# Autodesk Inventor assembly: full_layout_test
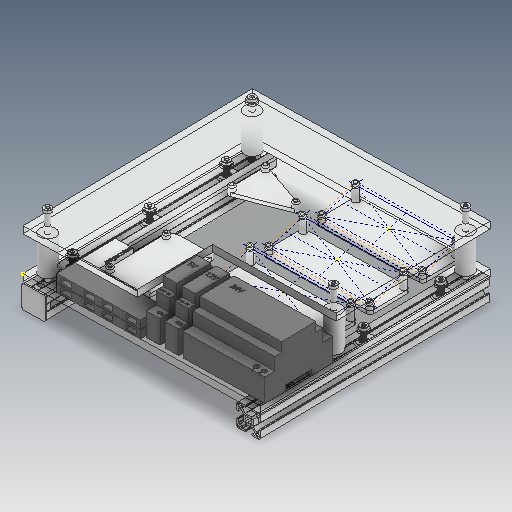
[picture p0: Inventor's stored thumbnail of the model, 512x512]
Saved by Autodesk Inventor 2025.4 (Build 294407020, 407B)
## iProperties
Created: 2026-09-08
Part Number: full_layout_test
Document SubType Name: Assembly
Designer: Aiden
Author: Aiden
## Documents named in this file (19)
- C:\Users\Aiden\Documents\GitHub\coldex-instrumentation\3d_models\mounting_hardware\dummy_parts\full_layout_test.iam
- C:\Users\Aiden\Documents\GitHub\coldex-instrumentation\3d_models\mounting_hardware\dummy_parts\acrylic_base.ipt
- C:\Users\Aiden\Documents\GitHub\coldex-instrumentation\3d_models\mounting_hardware\dummy_parts\acrylic_cover.ipt
- C:\Users\Aiden\Documents\GitHub\coldex-instrumentation\3d_models\mounting_hardware\McMaster\30mm_1ft_T-Slotted Framing.ipt
- C:\Users\Aiden\Documents\GitHub\coldex-instrumentation\3d_models\mounting_hardware\McMaster\30mm_teenut_T-Slotted Framing.ipt
- C:\Users\Aiden\Documents\GitHub\coldex-instrumentation\3d_models\mounting_hardware\McMaster\0.257in_innerD_Moisture-Resistant Cushioning Washer.ipt
- C:\Users\Aiden\Documents\GitHub\coldex-instrumentation\3d_models\mounting_hardware\McMaster\m6_18mm_18-8 Stainless Steel Low-Profile Socket Head Screws.ipt
- C:\Users\Aiden\Documents\GitHub\coldex-instrumentation\3d_models\mounting_hardware\dummy_parts\din_rail.ipt
- C:\Users\Aiden\Documents\GitHub\coldex-instrumentation\3d_models\mounting_hardware\dummy_parts\5V_din_voltage_regulator.ipt
- C:\Users\Aiden\Documents\GitHub\coldex-instrumentation\3d_models\mounting_hardware\dummy_parts\12V_din_voltage_regulator.ipt
- C:\Users\Aiden\Documents\GitHub\coldex-instrumentation\3d_models\mounting_hardware\dummy_parts\24V_din_pwr_supply.ipt
- C:\Users\Aiden\Documents\GitHub\coldex-instrumentation\3d_models\mounting_hardware\relay_module_standoffs_angled_plate.ipt
- C:\Users\Aiden\Documents\GitHub\coldex-instrumentation\3d_models\mounting_hardware\arduino_mega_standoffs_plate.ipt
- C:\Users\Aiden\Documents\GitHub\coldex-instrumentation\3d_models\mounting_hardware\dummy_parts\adalogger_mcu_volume.ipt
- C:\Users\Aiden\Documents\GitHub\coldex-instrumentation\3d_models\mounting_hardware\db-25_standoffs_plate.ipt
- C:\Users\Aiden\Documents\GitHub\coldex-instrumentation\3d_models\mounting_hardware\dummy_parts\anker_4-port_usb3.0_splitter.ipt
- C:\Users\Aiden\Documents\GitHub\coldex-instrumentation\3d_models\mounting_hardware\dummy_parts\spacer_temp.ipt
- C:\Users\Aiden\Documents\GitHub\coldex-instrumentation\3d_models\mounting_hardware\McMaster\m6_70mm_18-8 Stainless Steel Low-Profile Socket Head Screws.ipt
- C:\Users\Aiden\Documents\GitHub\coldex-instrumentation\3d_models\mounting_hardware\dummy_parts\8020_Cap.ipt
## Components (44 placed, 18 different names)
1. acrylic_base:1 — Flush:1, Flush:2, Mate:1, Mate:2, Flush:3, Flush:4, Mate:9, Mate:10, Mate:11, Mate:12, Mate:13, Mate:14, Mate:21, Mate:22, Mate:23, Mate:24, Mate:25, Mate:26, Mate:39, Mate:47, Angle:1, Flush:6, Mate:48, Angle:2, Angle:3, Mate:49, Mate:50, Angle:4, Mate:51, Flush:7, Mate:53, Mate:54, Mate:55, Mate:56, Mate:57, Mate:58, Mate:59, Mate:60
2. acrylic_cover:1 — Flush:1, Flush:2, Mate:61, Mate:62, Mate:63, Mate:64, Mate:65, Mate:67
3. 30mm_1ft_T-Slotted Framing:1 — Mate:1, Flush:4, Mate:3, Mate:4, Mate:5, Tangent:2, Flush:10
4. 30mm_1ft_T-Slotted Framing:2 — Mate:2, Flush:3, Mate:6, Mate:7, Mate:8, Tangent:1, Flush:5
5. 30mm_teenut_T-Slotted Framing:1 — Mate:5, Mate:9
6. 30mm_teenut_T-Slotted Framing:2 — Mate:3, Mate:10
7. 30mm_teenut_T-Slotted Framing:3 — Mate:4, Mate:11, Tangent:2
8. 30mm_teenut_T-Slotted Framing:4 — Mate:7, Mate:13
9. 30mm_teenut_T-Slotted Framing:5 — Mate:6, Mate:14
10. 30mm_teenut_T-Slotted Framing:6 — Mate:8, Mate:12, Tangent:1
11. m6_18mm_18-8 Stainless Steel Low-Profile Socket Head Screws:1 — Mate:35
12. m6_18mm_18-8 Stainless Steel Low-Profile Socket Head Screws:2 — Mate:34
13. m6_18mm_18-8 Stainless Steel Low-Profile Socket Head Screws:3
14. m6_18mm_18-8 Stainless Steel Low-Profile Socket Head Screws:4 — Mate:36
15. m6_18mm_18-8 Stainless Steel Low-Profile Socket Head Screws:5 — Mate:37
16. m6_18mm_18-8 Stainless Steel Low-Profile Socket Head Screws:6 — Mate:38, Mate:40
17. 0.257in_innerD_Moisture-Resistant Cushioning Washer:1 — Mate:22, Mate:34
18. 0.257in_innerD_Moisture-Resistant Cushioning Washer:2 — Mate:23, Mate:35
19. 0.257in_innerD_Moisture-Resistant Cushioning Washer:3 — Mate:24, Mate:38
20. 0.257in_innerD_Moisture-Resistant Cushioning Washer:4 — Mate:26, Mate:36
21. 0.257in_innerD_Moisture-Resistant Cushioning Washer:5 — Mate:25, Mate:37
22. 0.257in_innerD_Moisture-Resistant Cushioning Washer:6 — Mate:21
23. din_rail:1 — Mate:39, Mate:40, Mate:41, Mate:42, Mate:43, Mate:44, Mate:45, Mate:46
24. 5V_din_voltage_regulator:1 — Mate:41, Mate:42
25. 12V_din_voltage_regulator:1 — Mate:43, Mate:44
26. 24V_din_pwr_supply:1 — Mate:45, Mate:46
27. arduino_mega_standoffs_plate:1 — Angle:3, Mate:49
28. adalogger_mcu_volume:1 — Mate:48, Angle:2
29. db-25_standoffs_plate:1 — Mate:50, Angle:4
30. anker_4-port_usb3.0_splitter:1 — Mate:51, Flush:7, Flush:8, Mate:52, Flush:9
31. anker_4-port_usb3.0_splitter:2 — Flush:8, Mate:52, Flush:9
32. spacer_temp:1 — Mate:53, Mate:58
33. spacer_temp:2 — Mate:54, Mate:60
34. spacer_temp:3 — Mate:56, Mate:59
35. spacer_temp:4 — Mate:55, Mate:57, Mate:61
36. m6_70mm_18-8 Stainless Steel Low-Profile Socket Head Screws:1 — Mate:62, Mate:66, Mate:68
37. m6_70mm_18-8 Stainless Steel Low-Profile Socket Head Screws:2 — Mate:63
38. m6_70mm_18-8 Stainless Steel Low-Profile Socket Head Screws:3 — Mate:64
39. m6_70mm_18-8 Stainless Steel Low-Profile Socket Head Screws:4 — Mate:65
40. 0.257in_innerD_Moisture-Resistant Cushioning Washer:7 — Mate:66, Mate:67, Mate:68
41. 8020_Cap:1 — Flush:10
42. relay_module_standoffs_angled_plate:1 — Mate:47, Angle:1, Flush:6
43. relay_module_standoffs_angled_plate:2 — Flush:5
44. relay_module_standoffs_angled_plate:3
## Component patterns: (3 elements, first: relay_module_standoffs_angled_plate:1)
## Relationships (84: Mate 68, Flush 10, Angle 4, Tangent 2)
- Flush:1: acrylic_base:1 ↔ acrylic_cover:1
- Flush:2: acrylic_base:1 ↔ acrylic_cover:1
- Mate:1: acrylic_base:1 ↔ 30mm_1ft_T-Slotted Framing:1
- Mate:2: acrylic_base:1 ↔ 30mm_1ft_T-Slotted Framing:2
- Flush:3: acrylic_base:1 ↔ 30mm_1ft_T-Slotted Framing:2
- Flush:4: acrylic_base:1 ↔ 30mm_1ft_T-Slotted Framing:1
- Mate:3: 30mm_1ft_T-Slotted Framing:1 ↔ 30mm_teenut_T-Slotted Framing:2
- Mate:4: 30mm_1ft_T-Slotted Framing:1 ↔ 30mm_teenut_T-Slotted Framing:3
- Mate:5: 30mm_1ft_T-Slotted Framing:1 ↔ 30mm_teenut_T-Slotted Framing:1
- Mate:6: 30mm_1ft_T-Slotted Framing:2 ↔ 30mm_teenut_T-Slotted Framing:5
- Mate:7: 30mm_1ft_T-Slotted Framing:2 ↔ 30mm_teenut_T-Slotted Framing:4
- Mate:8: 30mm_1ft_T-Slotted Framing:2 ↔ 30mm_teenut_T-Slotted Framing:6
- Mate:9: acrylic_base:1 ↔ 30mm_teenut_T-Slotted Framing:1
- Mate:10: acrylic_base:1 ↔ 30mm_teenut_T-Slotted Framing:2
- Mate:11: acrylic_base:1 ↔ 30mm_teenut_T-Slotted Framing:3
- Mate:12: acrylic_base:1 ↔ 30mm_teenut_T-Slotted Framing:6
- Mate:13: acrylic_base:1 ↔ 30mm_teenut_T-Slotted Framing:4
- Mate:14: acrylic_base:1 ↔ 30mm_teenut_T-Slotted Framing:5
- Tangent:1: 30mm_1ft_T-Slotted Framing:2 ↔ 30mm_teenut_T-Slotted Framing:6
- Tangent:2: 30mm_1ft_T-Slotted Framing:1 ↔ 30mm_teenut_T-Slotted Framing:3
- [Mate]: acrylic_base:1 ↔ m6_18mm_18-8 Stainless Steel Low-Profile Socket Head Screws:1
- [Mate]: acrylic_base:1 ↔ m6_18mm_18-8 Stainless Steel Low-Profile Socket Head Screws:2
- [Mate]: acrylic_base:1 ↔ m6_18mm_18-8 Stainless Steel Low-Profile Socket Head Screws:3
- [Mate]: acrylic_base:1 ↔ m6_18mm_18-8 Stainless Steel Low-Profile Socket Head Screws:4
- [Mate]: acrylic_base:1 ↔ m6_18mm_18-8 Stainless Steel Low-Profile Socket Head Screws:5
- [Mate]: acrylic_base:1 ↔ m6_18mm_18-8 Stainless Steel Low-Profile Socket Head Screws:6
- Mate:21: acrylic_base:1 ↔ 0.257in_innerD_Moisture-Resistant Cushioning Washer:6
- Mate:22: acrylic_base:1 ↔ 0.257in_innerD_Moisture-Resistant Cushioning Washer:1
- Mate:23: acrylic_base:1 ↔ 0.257in_innerD_Moisture-Resistant Cushioning Washer:2
- Mate:24: acrylic_base:1 ↔ 0.257in_innerD_Moisture-Resistant Cushioning Washer:3
- Mate:25: acrylic_base:1 ↔ 0.257in_innerD_Moisture-Resistant Cushioning Washer:5
- Mate:26: acrylic_base:1 ↔ 0.257in_innerD_Moisture-Resistant Cushioning Washer:4
- [Mate]: m6_18mm_18-8 Stainless Steel Low-Profile Socket Head Screws:3 ↔ 0.257in_innerD_Moisture-Resistant Cushioning Washer:6
- [Mate]: m6_18mm_18-8 Stainless Steel Low-Profile Socket Head Screws:2 ↔ 0.257in_innerD_Moisture-Resistant Cushioning Washer:1
- [Mate]: m6_18mm_18-8 Stainless Steel Low-Profile Socket Head Screws:1 ↔ 0.257in_innerD_Moisture-Resistant Cushioning Washer:2
- [Mate]: m6_18mm_18-8 Stainless Steel Low-Profile Socket Head Screws:6 ↔ 0.257in_innerD_Moisture-Resistant Cushioning Washer:3
- [Mate]: m6_18mm_18-8 Stainless Steel Low-Profile Socket Head Screws:5 ↔ 0.257in_innerD_Moisture-Resistant Cushioning Washer:5
- [Mate]: m6_18mm_18-8 Stainless Steel Low-Profile Socket Head Screws:4 ↔ 0.257in_innerD_Moisture-Resistant Cushioning Washer:4
- [Mate]: m6_18mm_18-8 Stainless Steel Low-Profile Socket Head Screws:3 ↔ 0.257in_innerD_Moisture-Resistant Cushioning Washer:6
- Mate:34: m6_18mm_18-8 Stainless Steel Low-Profile Socket Head Screws:2 ↔ 0.257in_innerD_Moisture-Resistant Cushioning Washer:1
- Mate:35: m6_18mm_18-8 Stainless Steel Low-Profile Socket Head Screws:1 ↔ 0.257in_innerD_Moisture-Resistant Cushioning Washer:2
- Mate:36: m6_18mm_18-8 Stainless Steel Low-Profile Socket Head Screws:4 ↔ 0.257in_innerD_Moisture-Resistant Cushioning Washer:4
- Mate:37: m6_18mm_18-8 Stainless Steel Low-Profile Socket Head Screws:5 ↔ 0.257in_innerD_Moisture-Resistant Cushioning Washer:5
- Mate:38: m6_18mm_18-8 Stainless Steel Low-Profile Socket Head Screws:6 ↔ 0.257in_innerD_Moisture-Resistant Cushioning Washer:3
- Mate:39: acrylic_base:1 ↔ din_rail:1
- Mate:40: m6_18mm_18-8 Stainless Steel Low-Profile Socket Head Screws:6 ↔ din_rail:1
- Mate:41: din_rail:1 ↔ 5V_din_voltage_regulator:1
- Mate:42: din_rail:1 ↔ 5V_din_voltage_regulator:1
- Mate:43: din_rail:1 ↔ 12V_din_voltage_regulator:1
- Mate:44: din_rail:1 ↔ 12V_din_voltage_regulator:1
- Mate:45: din_rail:1 ↔ 24V_din_pwr_supply:1
- Mate:46: din_rail:1 ↔ 24V_din_pwr_supply:1
- Mate:47: acrylic_base:1 ↔ relay_module_standoffs_angled_plate:1
- Angle:1 (0 deg): acrylic_base:1 ↔ relay_module_standoffs_angled_plate:1
- Flush:5 (27 mm): 30mm_1ft_T-Slotted Framing:2 ↔ relay_module_standoffs_angled_plate:2
- Flush:6 (7.5 mm): acrylic_base:1 ↔ relay_module_standoffs_angled_plate:1
- Mate:48: acrylic_base:1 ↔ adalogger_mcu_volume:1
- Angle:2 (0 deg): acrylic_base:1 ↔ adalogger_mcu_volume:1
- Angle:3 (0 deg): acrylic_base:1 ↔ arduino_mega_standoffs_plate:1
- Mate:49: acrylic_base:1 ↔ arduino_mega_standoffs_plate:1
- Mate:50: acrylic_base:1 ↔ db-25_standoffs_plate:1
- Angle:4 (0 deg): acrylic_base:1 ↔ db-25_standoffs_plate:1
- Mate:51: acrylic_base:1 ↔ anker_4-port_usb3.0_splitter:1
- Flush:7: acrylic_base:1 ↔ anker_4-port_usb3.0_splitter:1
- Flush:8: anker_4-port_usb3.0_splitter:1 ↔ anker_4-port_usb3.0_splitter:2
- Mate:52 (1 mm): anker_4-port_usb3.0_splitter:1 ↔ anker_4-port_usb3.0_splitter:2
- Flush:9: anker_4-port_usb3.0_splitter:1 ↔ anker_4-port_usb3.0_splitter:2
- Mate:53: acrylic_base:1 ↔ spacer_temp:1
- Mate:54: acrylic_base:1 ↔ spacer_temp:2
- Mate:55: acrylic_base:1 ↔ spacer_temp:4
- Mate:56: acrylic_base:1 ↔ spacer_temp:3
- Mate:57: acrylic_base:1 ↔ spacer_temp:4
- Mate:58: acrylic_base:1 ↔ spacer_temp:1
- Mate:59: acrylic_base:1 ↔ spacer_temp:3
- Mate:60: acrylic_base:1 ↔ spacer_temp:2
- Mate:61: acrylic_cover:1 ↔ spacer_temp:4
- Mate:62: acrylic_cover:1 ↔ m6_70mm_18-8 Stainless Steel Low-Profile Socket Head Screws:1
- Mate:63: acrylic_cover:1 ↔ m6_70mm_18-8 Stainless Steel Low-Profile Socket Head Screws:2
- Mate:64: acrylic_cover:1 ↔ m6_70mm_18-8 Stainless Steel Low-Profile Socket Head Screws:3
- Mate:65: acrylic_cover:1 ↔ m6_70mm_18-8 Stainless Steel Low-Profile Socket Head Screws:4
- Mate:66: m6_70mm_18-8 Stainless Steel Low-Profile Socket Head Screws:1 ↔ 0.257in_innerD_Moisture-Resistant Cushioning Washer:7
- Mate:67: acrylic_cover:1 ↔ 0.257in_innerD_Moisture-Resistant Cushioning Washer:7
- Mate:68: m6_70mm_18-8 Stainless Steel Low-Profile Socket Head Screws:1 ↔ 0.257in_innerD_Moisture-Resistant Cushioning Washer:7
- Flush:10: 30mm_1ft_T-Slotted Framing:1 ↔ 8020_Cap:1
